# Autodesk Inventor assembly: HammerStick Hook1
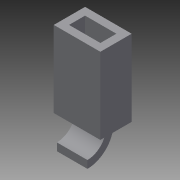
[picture p0: Inventor's stored thumbnail of the model, 180x180]
Saved by Autodesk Inventor 2015 (Build 190159000, 159)
## iProperties
Created: 2015-01-13
Part Number: HammerStick Hook1
Document SubType Name: Assembly
Designer: harrykuperstein
Author: harrykuperstein
## Documents named in this file (3)
- C:\team3556-cad-2015\HammerStick Hook1.iam
- C:\team3556-cad-2015\HammerStick Hook.ipt
- C:\team3556-cad-2015\HammerStick Sleeve.ipt
## Components (2 placed, 2 different names)
1. HammerStick Hook:1 — Mate:1, Tangent:1, Flush:1
2. HammerStick Sleeve:1 — Mate:1, Tangent:1, Flush:1
## Relationships (3: Mate 1, Tangent 1, Flush 1)
- Mate:1: HammerStick Hook:1 ↔ HammerStick Sleeve:1
- Tangent:1 (17.78 mm): HammerStick Hook:1 ↔ HammerStick Sleeve:1
- Flush:1 (-14.224 mm): HammerStick Hook:1 ↔ HammerStick Sleeve:1
